# Autodesk Inventor assembly: tmp_chain
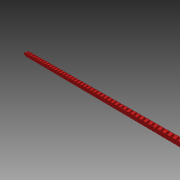
[picture p0: Inventor's stored thumbnail of the model, 180x180]
Saved by Autodesk Inventor 2014 (Build 180170000, 170)
## iProperties
Created: 2014-01-11
Part Number: tmp_chain
Document SubType Name: Assembly
Designer: buben
Author: buben
## Documents named in this file (2)
- C:\Users\buben\Documents\GitHub\bacon\inventor files\utils\tmp_chain.iam
- C:\Users\buben\Documents\GitHub\bacon\inventor files\utils\cable_chain_22.ipt
## Components (48 placed, 1 different names)
1. cable_chain_22:1 — Mate:1, Mate:2, Mate:3, Insert:1, Angle:1
2. cable_chain_22:2 — Insert:1, Angle:1, Insert:2, Angle:2
3. cable_chain_22:3 — Insert:2, Angle:2, Insert:5, Angle:5
4. cable_chain_22:4 — Insert:5, Angle:5
5. cable_chain_22:5
6. cable_chain_22:6 — Insert:11, Angle:11
7. cable_chain_22:7 — Insert:11, Angle:11
8. cable_chain_22:8
9. cable_chain_22:9
10. cable_chain_22:10
11. cable_chain_22:11
12. cable_chain_22:12 — Insert:23, Angle:23
13. cable_chain_22:13 — Insert:23, Angle:23
14. cable_chain_22:14
15. cable_chain_22:15
16. cable_chain_22:16
17. cable_chain_22:17
18. cable_chain_22:18
19. cable_chain_22:19
20. cable_chain_22:20
21. cable_chain_22:21
22. cable_chain_22:22
23. cable_chain_22:23
24. cable_chain_22:24 — Insert:47, Angle:47
25. cable_chain_22:25 — Insert:47, Angle:47
26. cable_chain_22:26
27. cable_chain_22:27
28. cable_chain_22:28
29. cable_chain_22:29
30. cable_chain_22:30
31. cable_chain_22:31
32. cable_chain_22:32
33. cable_chain_22:33
34. cable_chain_22:34
35. cable_chain_22:35
36. cable_chain_22:36
37. cable_chain_22:37
38. cable_chain_22:38
39. cable_chain_22:39
40. cable_chain_22:40
41. cable_chain_22:41
42. cable_chain_22:42
43. cable_chain_22:43
44. cable_chain_22:44
45. cable_chain_22:45
46. cable_chain_22:46
47. cable_chain_22:47
48. cable_chain_22:48
## Relationships (97: Insert 47, Angle 47, Mate 3)
- Mate:1: cable_chain_22:1
- Mate:2: cable_chain_22:1
- Mate:3: cable_chain_22:1
- Insert:1: cable_chain_22:1 ↔ cable_chain_22:2
- Angle:1 (-36 deg): cable_chain_22:1 ↔ cable_chain_22:2
- Insert:2: cable_chain_22:2 ↔ cable_chain_22:3
- Angle:2 (-36 deg): cable_chain_22:2 ↔ cable_chain_22:3
- [Insert]: cable_chain_22:4 ↔ cable_chain_22:5
- [Angle] (-36 deg): cable_chain_22:4 ↔ cable_chain_22:5
- [Insert]: cable_chain_22:5 ↔ cable_chain_22:6
- [Angle] (-36 deg): cable_chain_22:5 ↔ cable_chain_22:6
- Insert:5: cable_chain_22:3 ↔ cable_chain_22:4
- Angle:5 (-36 deg): cable_chain_22:3 ↔ cable_chain_22:4
- [Insert]: cable_chain_22:7 ↔ cable_chain_22:8
- [Angle] (-36 deg): cable_chain_22:7 ↔ cable_chain_22:8
- [Insert]: cable_chain_22:8 ↔ cable_chain_22:9
- [Angle] (-36 deg): cable_chain_22:8 ↔ cable_chain_22:9
- [Insert]: cable_chain_22:10 ↔ cable_chain_22:11
- [Angle] (-36 deg): cable_chain_22:10 ↔ cable_chain_22:11
- [Insert]: cable_chain_22:11 ↔ cable_chain_22:12
- [Angle] (-36 deg): cable_chain_22:11 ↔ cable_chain_22:12
- [Insert]: cable_chain_22:9 ↔ cable_chain_22:10
- [Angle] (-36 deg): cable_chain_22:9 ↔ cable_chain_22:10
- Insert:11: cable_chain_22:6 ↔ cable_chain_22:7
- Angle:11 (-36 deg): cable_chain_22:6 ↔ cable_chain_22:7
- [Insert]: cable_chain_22:13 ↔ cable_chain_22:14
- [Angle] (-36 deg): cable_chain_22:13 ↔ cable_chain_22:14
- [Insert]: cable_chain_22:14 ↔ cable_chain_22:15
- [Angle] (-36 deg): cable_chain_22:14 ↔ cable_chain_22:15
- [Insert]: cable_chain_22:16 ↔ cable_chain_22:17
- [Angle] (-36 deg): cable_chain_22:16 ↔ cable_chain_22:17
- [Insert]: cable_chain_22:17 ↔ cable_chain_22:18
- [Angle] (-36 deg): cable_chain_22:17 ↔ cable_chain_22:18
- [Insert]: cable_chain_22:15 ↔ cable_chain_22:16
- [Angle] (-36 deg): cable_chain_22:15 ↔ cable_chain_22:16
- [Insert]: cable_chain_22:19 ↔ cable_chain_22:20
- [Angle] (-36 deg): cable_chain_22:19 ↔ cable_chain_22:20
- [Insert]: cable_chain_22:20 ↔ cable_chain_22:21
- [Angle] (-36 deg): cable_chain_22:20 ↔ cable_chain_22:21
- [Insert]: cable_chain_22:22 ↔ cable_chain_22:23
- [Angle] (-36 deg): cable_chain_22:22 ↔ cable_chain_22:23
- [Insert]: cable_chain_22:23 ↔ cable_chain_22:24
- [Angle] (-36 deg): cable_chain_22:23 ↔ cable_chain_22:24
- [Insert]: cable_chain_22:21 ↔ cable_chain_22:22
- [Angle] (-36 deg): cable_chain_22:21 ↔ cable_chain_22:22
- [Insert]: cable_chain_22:18 ↔ cable_chain_22:19
- [Angle] (-36 deg): cable_chain_22:18 ↔ cable_chain_22:19
- Insert:23: cable_chain_22:12 ↔ cable_chain_22:13
- Angle:23 (-36 deg): cable_chain_22:12 ↔ cable_chain_22:13
- [Insert]: cable_chain_22:25 ↔ cable_chain_22:26
- [Angle] (-36 deg): cable_chain_22:25 ↔ cable_chain_22:26
- [Insert]: cable_chain_22:26 ↔ cable_chain_22:27
- [Angle] (-36 deg): cable_chain_22:26 ↔ cable_chain_22:27
- [Insert]: cable_chain_22:28 ↔ cable_chain_22:29
- [Angle] (-36 deg): cable_chain_22:28 ↔ cable_chain_22:29
- [Insert]: cable_chain_22:29 ↔ cable_chain_22:30
- [Angle] (-36 deg): cable_chain_22:29 ↔ cable_chain_22:30
- [Insert]: cable_chain_22:27 ↔ cable_chain_22:28
- [Angle] (-36 deg): cable_chain_22:27 ↔ cable_chain_22:28
- [Insert]: cable_chain_22:31 ↔ cable_chain_22:32
- [Angle] (-36 deg): cable_chain_22:31 ↔ cable_chain_22:32
- [Insert]: cable_chain_22:32 ↔ cable_chain_22:33
- [Angle] (-36 deg): cable_chain_22:32 ↔ cable_chain_22:33
- [Insert]: cable_chain_22:34 ↔ cable_chain_22:35
- [Angle] (-36 deg): cable_chain_22:34 ↔ cable_chain_22:35
- [Insert]: cable_chain_22:35 ↔ cable_chain_22:36
- [Angle] (-36 deg): cable_chain_22:35 ↔ cable_chain_22:36
- [Insert]: cable_chain_22:33 ↔ cable_chain_22:34
- [Angle] (-36 deg): cable_chain_22:33 ↔ cable_chain_22:34
- [Insert]: cable_chain_22:30 ↔ cable_chain_22:31
- [Angle] (-36 deg): cable_chain_22:30 ↔ cable_chain_22:31
- [Insert]: cable_chain_22:37 ↔ cable_chain_22:38
- [Angle] (-36 deg): cable_chain_22:37 ↔ cable_chain_22:38
- [Insert]: cable_chain_22:38 ↔ cable_chain_22:39
- [Angle] (-36 deg): cable_chain_22:38 ↔ cable_chain_22:39
- [Insert]: cable_chain_22:40 ↔ cable_chain_22:41
- [Angle] (-36 deg): cable_chain_22:40 ↔ cable_chain_22:41
- [Insert]: cable_chain_22:41 ↔ cable_chain_22:42
- [Angle] (-36 deg): cable_chain_22:41 ↔ cable_chain_22:42
- [Insert]: cable_chain_22:39 ↔ cable_chain_22:40
- [Angle] (-36 deg): cable_chain_22:39 ↔ cable_chain_22:40
- [Insert]: cable_chain_22:43 ↔ cable_chain_22:44
- [Angle] (-36 deg): cable_chain_22:43 ↔ cable_chain_22:44
- [Insert]: cable_chain_22:44 ↔ cable_chain_22:45
- [Angle] (-36 deg): cable_chain_22:44 ↔ cable_chain_22:45
- [Insert]: cable_chain_22:46 ↔ cable_chain_22:47
- [Angle] (-36 deg): cable_chain_22:46 ↔ cable_chain_22:47
- [Insert]: cable_chain_22:47 ↔ cable_chain_22:48
- [Angle] (-36 deg): cable_chain_22:47 ↔ cable_chain_22:48
- [Insert]: cable_chain_22:45 ↔ cable_chain_22:46
- [Angle] (-36 deg): cable_chain_22:45 ↔ cable_chain_22:46
- [Insert]: cable_chain_22:42 ↔ cable_chain_22:43
- [Angle] (-36 deg): cable_chain_22:42 ↔ cable_chain_22:43
- [Insert]: cable_chain_22:36 ↔ cable_chain_22:37
- [Angle] (-36 deg): cable_chain_22:36 ↔ cable_chain_22:37
- Insert:47: cable_chain_22:24 ↔ cable_chain_22:25
- Angle:47 (-36 deg): cable_chain_22:24 ↔ cable_chain_22:25
## Named parameters: d392_d389 = -36 deg, d393_d390 = 0 deg, d394_d391 = -36 deg, d395_d382 = 0 mm, d396_d383 = -36 deg, d397_d384 = 0 deg, d398_d385 = -36 deg, d399_d386 = 0 mm, d400_d387 = 0 mm, d401_d388 = 0 mm, d406_d403 = -36 deg, d407_d404 = 0 deg, d408_d405 = -36 deg, d409_d389 = -36 deg, d410_d390 = 0 deg, d411_d391 = -36 deg, d412_d392_d389 = -36 deg, d413_d393_d390 = 0 deg, d414_d394_d391 = -36 deg, d415_d395_d382 = 0 mm, d416_d396_d383 = -36 deg, d417_d397_d384 = 0 deg, d418_d398_d385 = -36 deg, d419_d399_d386 = 0 mm, d420_d400_d387 = 0 mm, d421_d401_d388 = 0 mm, d422_d402 = 0 mm, d423_d382 = 0 mm, d424_d383 = -36 deg, d425_d384 = 0 deg, d426_d385 = -36 deg, d427_d386 = 0 mm, d428_d387 = 0 mm, d429_d388 = 0 mm, d434_d431 = -36 deg, d435_d432 = 0 deg, d436_d433 = -36 deg, d437_d403 = -36 deg, d438_d404 = 0 deg, d439_d405 = -36 deg, d440_d406_d403 = -36 deg, d441_d407_d404 = 0 deg, d442_d408_d405 = -36 deg, d443_d409_d389 = -36 deg, d444_d410_d390 = 0 deg, d445_d411_d391 = -36 deg, d446_d412_d392_d389 = -36 deg, d447_d413_d393_d390 = 0 deg, d448_d414_d394_d391 = -36 deg, d449_d415_d395_d382 = 0 mm, d450_d416_d396_d383 = -36 deg, d451_d417_d397_d384 = 0 deg, d452_d418_d398_d385 = -36 deg, d453_d419_d399_d386 = 0 mm, d454_d420_d400_d387 = 0 mm, d455_d421_d401_d388 = 0 mm, d456_d422_d402 = 0 mm, d457_d423_d382 = 0 mm, d458_d424_d383 = -36 deg, d459_d425_d384 = 0 deg, d460_d426_d385 = -36 deg, d461_d427_d386 = 0 mm, d462_d428_d387 = 0 mm, d463_d429_d388 = 0 mm, d464_d430 = 0 mm, d465_d389 = -36 deg, d466_d390 = 0 deg, d467_d391 = -36 deg, d468_d392_d389 = -36 deg, d469_d393_d390 = 0 deg, d470_d394_d391 = -36 deg, d471_d395_d382 = 0 mm, d472_d396_d383 = -36 deg, d473_d397_d384 = 0 deg, d474_d398_d385 = -36 deg, d475_d399_d386 = 0 mm, d476_d400_d387 = 0 mm, d477_d401_d388 = 0 mm, d478_d402 = 0 mm, d479_d382 = 0 mm, d480_d383 = -36 deg, d481_d384 = 0 deg, d482_d385 = -36 deg, d483_d386 = 0 mm, d484_d387 = 0 mm, d485_d388 = 0 mm, d490_d486 = 0 mm, d491_d487 = -36 deg, d492_d488 = 0 deg, d493_d489 = -36 deg, d494_d431 = -36 deg, d495_d432 = 0 deg, d496_d433 = -36 deg, d497_d434_d431 = -36 deg, d498_d435_d432 = 0 deg, d499_d436_d433 = -36 deg, d500_d437_d403 = -36 deg, d501_d438_d404 = 0 deg, d502_d439_d405 = -36 deg, d503_d440_d406_d403 = -36 deg, d504_d441_d407_d404 = 0 deg, d505_d442_d408_d405 = -36 deg, d506_d443_d409_d389 = -36 deg, d507_d444_d410_d390 = 0 deg, d508_d445_d411_d391 = -36 deg, d509_d446_d412_d392_d389 = -36 deg, d510_d447_d413_d393_d390 = 0 deg, d511_d448_d414_d394_d391 = -36 deg, d512_d449_d415_d395_d382 = 0 mm, d513_d450_d416_d396_d383 = -36 deg, d514_d451_d417_d397_d384 = 0 deg, d515_d452_d418_d398_d385 = -36 deg, d516_d453_d419_d399_d386 = 0 mm, d517_d454_d420_d400_d387 = 0 mm, d518_d455_d421_d401_d388 = 0 mm, d519_d456_d422_d402 = 0 mm, d520_d457_d423_d382 = 0 mm, d521_d458_d424_d383 = -36 deg, d522_d459_d425_d384 = 0 deg, d523_d460_d426_d385 = -36 deg, d524_d461_d427_d386 = 0 mm, d525_d462_d428_d387 = 0 mm, d526_d463_d429_d388 = 0 mm, d527_d464_d430 = 0 mm, d528_d465_d389 = -36 deg, d529_d466_d390 = 0 deg, d530_d467_d391 = -36 deg, d531_d468_d392_d389 = -36 deg, d532_d469_d393_d390 = 0 deg, d533_d470_d394_d391 = -36 deg, d534_d471_d395_d382 = 0 mm, d535_d472_d396_d383 = -36 deg, d536_d473_d397_d384 = 0 deg, d537_d474_d398_d385 = -36 deg, d538_d475_d399_d386 = 0 mm, d539_d476_d400_d387 = 0 mm, d540_d477_d401_d388 = 0 mm, d541_d478_d402 = 0 mm, d542_d479_d382 = 0 mm, d543_d480_d383 = -36 deg, d544_d481_d384 = 0 deg, d545_d482_d385 = -36 deg, d546_d483_d386 = 0 mm, d547_d484_d387 = 0 mm, d548_d485_d388 = 0 mm, d549_d403 = -36 deg, d550_d404 = 0 deg, d551_d405 = -36 deg, d552_d406_d403 = -36 deg, d553_d407_d404 = 0 deg, d554_d408_d405 = -36 deg, d555_d409_d389 = -36 deg, d556_d410_d390 = 0 deg, d557_d411_d391 = -36 deg, d558_d412_d392_d389 = -36 deg, d559_d413_d393_d390 = 0 deg, d560_d414_d394_d391 = -36 deg, d561_d415_d395_d382 = 0 mm, d562_d416_d396_d383 = -36 deg, d563_d417_d397_d384 = 0 deg, d564_d418_d398_d385 = -36 deg, d565_d419_d399_d386 = 0 mm, d566_d420_d400_d387 = 0 mm, d567_d421_d401_d388 = 0 mm, d568_d422_d402 = 0 mm, d569_d423_d382 = 0 mm, d570_d424_d383 = -36 deg, d571_d425_d384 = 0 deg, d572_d426_d385 = -36 deg, d573_d427_d386 = 0 mm, d574_d428_d387 = 0 mm, d575_d429_d388 = 0 mm, d576_d430 = 0 mm, d577_d389 = -36 deg, d578_d390 = 0 deg, d579_d391 = -36 deg, d580_d392_d389 = -36 deg, d581_d393_d390 = 0 deg, d582_d394_d391 = -36 deg, d583_d395_d382 = 0 mm, d584_d396_d383 = -36 deg, d585_d397_d384 = 0 deg, d586_d398_d385 = -36 deg, d587_d399_d386 = 0 mm, d588_d400_d387 = 0 mm, d589_d401_d388 = 0 mm, d590_d402 = 0 mm, d591_d382 = 0 mm, d592_d383 = -36 deg, d593_d384 = 0 deg, d594_d385 = -36 deg, d595_d386 = 0 mm, d596_d387 = 0 mm, d597_d388 = 0 mm
